# Autodesk Inventor assembly: S3x1
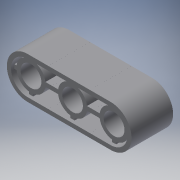
[picture p0: Inventor's stored thumbnail of the model, 180x180]
Saved by Autodesk Inventor 2019 (Build 230136000, 136)
## iProperties
Created: 2019-01-31
Part Number: S3x1
Document SubType Name: Assembly
Designer: Varga Daniel
Author: Varga Daniel
## Documents named in this file (4)
- C:\!_Dani\!_cloud\OneDrive\!_munka\Revolution\RevvyDemoKit\Structural parts\Straight Beams\S3+x1\S3x1.iam
- C:\!_Dani\!_cloud\OneDrive\!_munka\Revolution\RevvyDemoKit\Structural parts\Straight Beams\straight_beam_single_end_part.ipt
- C:\!_Dani\!_cloud\OneDrive\!_munka\Revolution\RevvyDemoKit\Structural parts\Straight Beams\straight_beam_single_inner_part.ipt
- C:\!_Dani\!_cloud\OneDrive\!_munka\Revolution\RevvyDemoKit\Structural parts\Straight Beams\S3+x1.iam
## Components (3 placed, 2 different names)
1. straight_beam_single_end_part:1 — Flush:1, Flush:2, Mate:1, Flush:3, Flush:4, Mate:2
2. straight_beam_single_end_part:2 — Flush:1, Flush:2, Mate:1
3. straight_beam_single_inner_part:1 — Flush:3, Flush:4, Mate:2
## Component patterns: (1 elements, first: straight_beam_single_inner_part:1)
## Relationships (6: Flush 4, Mate 2)
- Flush:1: straight_beam_single_end_part:1 ↔ straight_beam_single_end_part:2
- Flush:2: straight_beam_single_end_part:1 ↔ straight_beam_single_end_part:2
- Mate:1 (10 mm): straight_beam_single_end_part:1 ↔ straight_beam_single_end_part:2
- Flush:3: straight_beam_single_end_part:1 ↔ straight_beam_single_inner_part:1
- Flush:4: straight_beam_single_end_part:1 ↔ straight_beam_single_inner_part:1
- Mate:2: straight_beam_single_end_part:1 ↔ straight_beam_single_inner_part:1
